# Autodesk Inventor assembly: Group
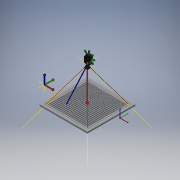
[picture p0: Inventor's stored thumbnail of the model, 180x180]
Saved by Autodesk Inventor 2018.2 (Build 222227000, 227)
## iProperties
Created: 2018-04-10
Part Number: Group
Material: Generisch
Document SubType Name: Assembly
Designer: Nick Koch
Author: Nick Koch
## Documents named in this file (9)
- C:\Users\Nick Koch\Desktop\Lehre\FHNW\Raytracing Modell\v5\Group.iam
- C:\Users\Nick Koch\Desktop\Lehre\FHNW\Raytracing Modell\v5\MiddleStick.ipt
- C:\Users\Nick Koch\Desktop\Lehre\FHNW\Raytracing Modell\v5\Camera.ipt
- C:\Users\Nick Koch\Desktop\Lehre\FHNW\Raytracing Modell\v5\blueStick.ipt
- C:\Users\Nick Koch\Desktop\Lehre\FHNW\Raytracing Modell\v5\FOVStick.ipt
- C:\Users\Nick Koch\Desktop\Lehre\FHNW\Raytracing Modell\v5\ArrowUp.ipt
- C:\Users\Nick Koch\Desktop\Lehre\FHNW\Raytracing Modell\v5\Screen2.ipt
- C:\Users\Nick Koch\Desktop\Lehre\FHNW\Raytracing Modell\v5\xyz_Axis.ipt
- C:\Users\Nick Koch\Desktop\Lehre\FHNW\Raytracing Modell\v5\Axis_Group.iam
## Components (15 placed, 8 different names)
1. MiddleStick:1 — Passend:4, Passend:5, Passend:6, Passend:48, Passend:49, Passend:50
2. Camera:1 — Passend:4, Passend:5, Passend:6, Passend:19, Passend:20, Passend:33, Passend:34, Passend:35, Passend:36, Passend:37, Passend:38, Passend:40, Passend:41, Passend:42, Passend:43, Passend:44, Passend:45, Passend:51, Passend:52, Passend:53, Passend:66, Passend:67, Passend:68
3. blueStick:3 — Passend:51, Passend:52, Passend:53
4. FOVStick:2 — Passend:60, Passend:61, Passend:62
5. FOVStick:3 — Passend:54, Passend:55, Passend:56
6. FOVStick:4 — Passend:57, Passend:58, Passend:59
7. FOVStick:5 — Passend:63, Passend:64, Passend:65
8. ArrowUp:1 — Passend:33, Passend:34, Passend:35
9. ArrowUp:2 — Passend:36, Passend:40, Passend:41
10. ArrowUp:3 — Passend:38, Passend:44, Passend:45
11. ArrowUp:5 — Passend:66, Passend:67, Passend:68
12. ArrowUp:6 — Passend:37, Passend:42, Passend:43
13. Screen2:1 — Passend:48, Passend:49, Passend:50, Passend:54, Passend:55, Passend:56, Passend:57, Passend:58, Passend:59, Passend:60, Passend:61, Passend:62, Passend:63, Passend:64, Passend:65
14. xyz_Axis:1
15. Axis_Group:1 [sub-assembly]
## Relationships (38: Mate 38)
- Passend:4 [Mate]: MiddleStick:1 ↔ Camera:1
- Passend:5 [Mate]: MiddleStick:1 ↔ Camera:1
- Passend:6 [Mate]: MiddleStick:1 ↔ Camera:1
- Passend:19 [Mate]: Camera:1
- Passend:20 [Mate]: Camera:1
- Passend:33 [Mate]: Camera:1 ↔ ArrowUp:1
- Passend:34 [Mate]: Camera:1 ↔ ArrowUp:1
- Passend:35 [Mate]: Camera:1 ↔ ArrowUp:1
- Passend:36 [Mate]: Camera:1 ↔ ArrowUp:2
- Passend:37 [Mate]: Camera:1 ↔ ArrowUp:6
- Passend:38 [Mate]: Camera:1 ↔ ArrowUp:3
- Passend:40 [Mate]: Camera:1 ↔ ArrowUp:2
- Passend:41 [Mate]: Camera:1 ↔ ArrowUp:2
- Passend:42 [Mate]: Camera:1 ↔ ArrowUp:6
- Passend:43 [Mate]: Camera:1 ↔ ArrowUp:6
- Passend:44 [Mate]: Camera:1 ↔ ArrowUp:3
- Passend:45 [Mate]: Camera:1 ↔ ArrowUp:3
- Passend:48 [Mate]: MiddleStick:1 ↔ Screen2:1
- Passend:49 [Mate]: MiddleStick:1 ↔ Screen2:1
- Passend:50 [Mate]: MiddleStick:1 ↔ Screen2:1
- Passend:51 [Mate]: Camera:1 ↔ blueStick:3
- Passend:52 [Mate]: Camera:1 ↔ blueStick:3
- Passend:53 [Mate]: Camera:1 ↔ blueStick:3
- Passend:54 [Mate]: FOVStick:3 ↔ Screen2:1
- Passend:55 [Mate]: FOVStick:3 ↔ Screen2:1
- Passend:56 [Mate]: FOVStick:3 ↔ Screen2:1
- Passend:57 [Mate]: FOVStick:4 ↔ Screen2:1
- Passend:58 [Mate]: FOVStick:4 ↔ Screen2:1
- Passend:59 [Mate]: FOVStick:4 ↔ Screen2:1
- Passend:60 [Mate]: FOVStick:2 ↔ Screen2:1
- Passend:61 [Mate]: FOVStick:2 ↔ Screen2:1
- Passend:62 [Mate]: FOVStick:2 ↔ Screen2:1
- Passend:63 [Mate]: FOVStick:5 ↔ Screen2:1
- Passend:64 [Mate]: FOVStick:5 ↔ Screen2:1
- Passend:65 [Mate]: FOVStick:5 ↔ Screen2:1
- Passend:66 [Mate]: Camera:1 ↔ ArrowUp:5
- Passend:67 [Mate]: Camera:1 ↔ ArrowUp:5
- Passend:68 [Mate]: Camera:1 ↔ ArrowUp:5
